# Autodesk Inventor assembly: Full Chassis with Arduino, Gyro, 1 inch Arms, and Flexiwheels
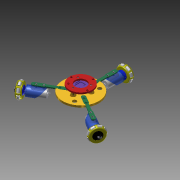
[picture p0: Inventor's stored thumbnail of the model, 180x180]
Saved by Autodesk Inventor 2014 (Build 180170000, 170)
## iProperties
Created: 2014-02-14
Part Number: Full Chassis with Arduino, Gyro, 1 inch Arms, and Flexiwheels
Document SubType Name: Assembly
Designer: Spooner
Author: Spooner
## Documents named in this file (3)
- C:\Users\Spooner\Documents\Inventor\FerretBall Robot\3Pod\Inventor 2014 Files\Full Chassis with Arduino, Gyro, 1 inch Arms, and Flexiwheels.iam
- C:\Users\Spooner\Documents\Inventor\FerretBall Robot\3Pod\Inventor 2014 Files\Main Body with Arduino and Gyro Mounts.iam
- C:\Users\Spooner\Documents\Inventor\FerretBall Robot\3Pod\Inventor 2014 Files\Full Motor Arm (1 inch) with Flexiwheel.iam
## Components (4 placed, 2 different names)
1. Main Body with Arduino and Gyro Mounts:1 [sub-assembly] — Insert:1, Mate:1, Insert:2, Mate:2, Insert:3, Mate:3
2. Full Motor Arm (1 inch) with Flexiwheel:1 [sub-assembly] — Insert:1, Mate:1
3. Full Motor Arm (1 inch) with Flexiwheel:2 [sub-assembly] — Insert:2, Mate:2
4. Full Motor Arm (1 inch) with Flexiwheel:3 [sub-assembly] — Insert:3, Mate:3
## Relationships (6: Insert 3, Mate 3)
- Insert:1: Main Body with Arduino and Gyro Mounts:1 ↔ Full Motor Arm (1 inch) with Flexiwheel:1
- Mate:1: Main Body with Arduino and Gyro Mounts:1 ↔ Full Motor Arm (1 inch) with Flexiwheel:1
- Insert:2: Main Body with Arduino and Gyro Mounts:1 ↔ Full Motor Arm (1 inch) with Flexiwheel:2
- Mate:2: Main Body with Arduino and Gyro Mounts:1 ↔ Full Motor Arm (1 inch) with Flexiwheel:2
- Insert:3: Main Body with Arduino and Gyro Mounts:1 ↔ Full Motor Arm (1 inch) with Flexiwheel:3
- Mate:3: Main Body with Arduino and Gyro Mounts:1 ↔ Full Motor Arm (1 inch) with Flexiwheel:3
